# Autodesk Inventor assembly: WashingMachineAssembly
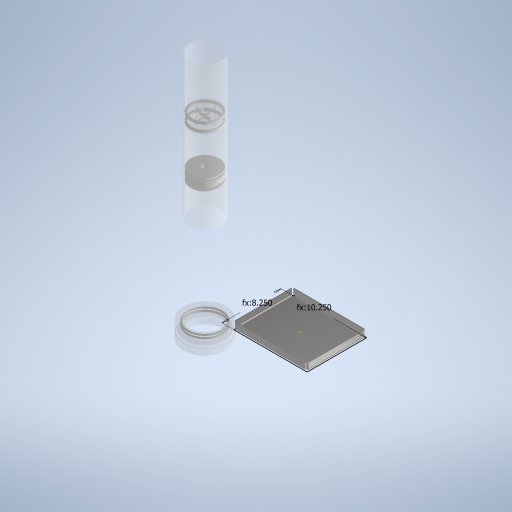
[picture p0: Inventor's stored thumbnail of the model, 512x512]
Saved by Autodesk Inventor 2024 (Build 280153000, 153)
## iProperties
Created: 2024-09-07
Part Number: WashingMachineAssembly
Document SubType Name: Assembly
Designer: Tommy Rohmann
Author: Tommy Rohmann
## Documents named in this file (11)
- C:\Users\Tommy Rohmann\OneDrive\Projects\Microgravity-Press-Washing-Machine\Inventor Design Project\WashingMachineAssembly.iam
- C:\Users\Tommy Rohmann\OneDrive\Projects\Microgravity-Press-Washing-Machine\Inventor Design Project\WashChamber.ipt
- C:\Users\Tommy Rohmann\OneDrive\Projects\Microgravity-Press-Washing-Machine\Inventor Design Project\PistonSeal.ipt
- C:\Users\Tommy Rohmann\OneDrive\Projects\Microgravity-Press-Washing-Machine\Inventor Design Project\ReserviorPiston.ipt
- C:\Users\Tommy Rohmann\OneDrive\Projects\Microgravity-Press-Washing-Machine\Inventor Design Project\RodSeal.ipt
- C:\Users\Tommy Rohmann\OneDrive\Projects\Microgravity-Press-Washing-Machine\Inventor Design Project\WashPiston.ipt
- C:\Users\Tommy Rohmann\OneDrive\Projects\Microgravity-Press-Washing-Machine\Inventor Design Project\WashChamberConduit.ipt
- C:\Users\Tommy Rohmann\OneDrive\Projects\Microgravity-Press-Washing-Machine\Inventor Design Project\FrameBase.ipt
- C:\Users\Tommy Rohmann\OneDrive\Projects\Microgravity-Press-Washing-Machine\Inventor Design Project\PistonStaticSeal.ipt
- C:\Users\Tommy Rohmann\OneDrive\Projects\Microgravity-Press-Washing-Machine\Inventor Design Project\WashChamberStaticSealConduit.ipt
- C:\Users\Tommy Rohmann\OneDrive\Projects\Microgravity-Press-Washing-Machine\Inventor Design Project\DesignParameters.xlsx
## Components (12 placed, 9 different names)
1. WashChamber:1 — Mate:12, Cylindrical:1, Cylindrical:2, Mate:14
2. PistonSeal:1 — Mate:7, Mate:8
3. PistonSeal:2 — Mate:1, Mate:2
4. ReserviorPiston:1 — Mate:1, Mate:2, Mate:3, Mate:4, Mate:5, Mate:6, Mate:7, Mate:8, Cylindrical:2
5. RodSeal:1 — Mate:3, Mate:4
6. RodSeal:2 — Mate:5, Mate:6
7. WashPiston:1 — Tangent:1, Mate:9, Cylindrical:1
8. FrameBase:1 — Flush:1, Mate:12
9. PistonStaticSeal:1 — Tangent:1, Mate:9
10. WashChamberStaticSealConduit:1 — Tangent:2, Mate:16
11. WashChamberConduit:1 — Mate:14, Tangent:2, Tangent:3, Mate:15, Mate:16
12. WashChamberStaticSealConduit:2 — Tangent:3, Mate:15
## Relationships (19: Mate 13, Tangent 3, CylindricalJoint 2, Flush 1)
- Mate:1: PistonSeal:2 ↔ ReserviorPiston:1
- Mate:2: PistonSeal:2 ↔ ReserviorPiston:1
- Mate:3: ReserviorPiston:1 ↔ RodSeal:1
- Mate:4: ReserviorPiston:1 ↔ RodSeal:1
- Mate:5: ReserviorPiston:1 ↔ RodSeal:2
- Mate:6: ReserviorPiston:1 ↔ RodSeal:2
- Mate:7: PistonSeal:1 ↔ ReserviorPiston:1
- Mate:8: PistonSeal:1 ↔ ReserviorPiston:1
- Flush:1: FrameBase:1
- Tangent:1: WashPiston:1 ↔ PistonStaticSeal:1
- Mate:9: WashPiston:1 ↔ PistonStaticSeal:1
- Mate:12: WashChamber:1 ↔ FrameBase:1
- Cylindrical:1: WashChamber:1 ↔ WashPiston:1
- Cylindrical:2: WashChamber:1 ↔ ReserviorPiston:1
- Mate:14: WashChamber:1 ↔ WashChamberConduit:1
- Tangent:2: WashChamberStaticSealConduit:1 ↔ WashChamberConduit:1
- Tangent:3: WashChamberConduit:1 ↔ WashChamberStaticSealConduit:2
- Mate:15: WashChamberConduit:1 ↔ WashChamberStaticSealConduit:2
- Mate:16: WashChamberStaticSealConduit:1 ↔ WashChamberConduit:1
## Named parameters: MachineMaxHeight = 539.75 mm, MachineMaxWidth = 215.9 mm, MachineMaxLength = 266.7 mm, MachineFluidCapacity = 25.4 mm, MaxCompressiveCapacity = 20320 mm, WashChamberID = 101.6 mm, WashChamberOD = 114.3 mm, SealedSurfaceOffset = 0.15875 mm, ConduitThickness = 152.4 mm, StaticORingThickness = 4.7625 mm
